# Autodesk Inventor assembly: Сборка2
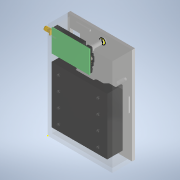
[picture p0: Inventor's stored thumbnail of the model, 180x180]
Saved by Autodesk Inventor 2022 (Build 260153000, 153)
## iProperties
Created: 2022-10-20
Part Number: Сборка2
Document SubType Name: Assembly
Designer: Robo0
Author: Robo0
## Documents named in this file (6)
- C:\Users\Robo0\Desktop\Новая папка\Сборка2.iam
- C:\Users\Robo0\Desktop\Новая папка\корпус.ipt
- C:\Users\Robo0\Desktop\Новая папка\Hold_18650-4.ipt
- C:\Users\Robo0\Desktop\Новая папка\goruntu modulu.ipt
- C:\Users\Robo0\Desktop\Новая папка\top.ipt
- C:\Users\Robo0\Desktop\Новая папка\butt.ipt
## Components (5 placed, 5 different names)
1. корпус:1 — Совмещение:1, Заподлицо:1, Заподлицо:2, Совмещение:3, Заподлицо:4, Заподлицо:5
2. Hold_18650-4:1 — Совмещение:1, Заподлицо:1, Заподлицо:2, Совмещение:2, Заподлицо:3
3. goruntu modulu:1 — Совмещение:2, Заподлицо:3, Совмещение:3, Совмещение:5
4. top:1 — Заподлицо:4, Заподлицо:5, Совмещение:4
5. butt:1 — Совмещение:4, Совмещение:5
## Relationships (10: Mate 5, Flush 5)
- Совмещение:1 [Mate]: корпус:1 ↔ Hold_18650-4:1
- Заподлицо:1 [Flush] (10 mm): корпус:1 ↔ Hold_18650-4:1
- Заподлицо:2 [Flush] (10 mm): корпус:1 ↔ Hold_18650-4:1
- Совмещение:2 [Mate] (10 mm): Hold_18650-4:1 ↔ goruntu modulu:1
- Заподлицо:3 [Flush]: Hold_18650-4:1 ↔ goruntu modulu:1
- Совмещение:3 [Mate]: корпус:1 ↔ goruntu modulu:1
- Заподлицо:4 [Flush]: корпус:1 ↔ top:1
- Заподлицо:5 [Flush]: корпус:1 ↔ top:1
- Совмещение:4 [Mate]: top:1 ↔ butt:1
- Совмещение:5 [Mate]: goruntu modulu:1 ↔ butt:1
